# Autodesk Inventor assembly: Pressure Vessel
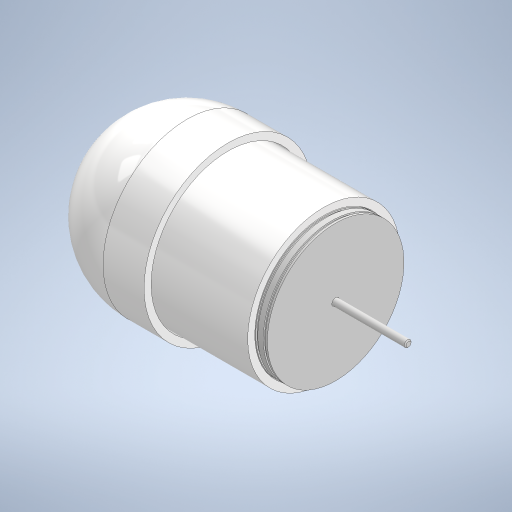
[picture p0: Inventor's stored thumbnail of the model, 512x512]
Saved by Autodesk Inventor 2023 (Build 270158030, 158C)
## iProperties
Created: 2022-09-17
Part Number: Pressure Vessel
Document SubType Name: Assembly
Designer: cjj5381
Author: cjj5381
## Documents named in this file (5)
- V:\Robtotics\Pressure Vessel.iam
- V:\Robtotics\PVC Pipe.ipt
- V:\Robtotics\Cap.ipt
- V:\Robtotics\Piston Head.ipt
- V:\Robtotics\92620A553_NO THREADS_Zinc Yellow-Chromate Plated Hex Head Screw.ipt
## Components (4 placed, 4 different names)
1. PVC Pipe:1 — Mate:1, Mate:2, Cylindrical:1
2. Cap:1 — Mate:1, Mate:2
3. Piston Head:1 — Mate:3, Mate:4, Cylindrical:1
4. 92620A553_NO THREADS_Zinc Yellow-Chromate Plated Hex Head Screw:1 — Mate:3, Mate:4
## Relationships (5: Mate 4, CylindricalJoint 1)
- Mate:1: PVC Pipe:1 ↔ Cap:1
- Mate:2: PVC Pipe:1 ↔ Cap:1
- Mate:3: Piston Head:1 ↔ 92620A553_NO THREADS_Zinc Yellow-Chromate Plated Hex Head Screw:1
- Mate:4: Piston Head:1 ↔ 92620A553_NO THREADS_Zinc Yellow-Chromate Plated Hex Head Screw:1
- Cylindrical:1: PVC Pipe:1 ↔ Piston Head:1
